# Autodesk Inventor assembly: PinBlock
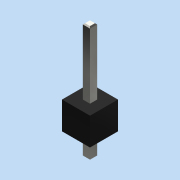
[picture p0: Inventor's stored thumbnail of the model, 180x180]
Saved by Autodesk Inventor 2017 (Build 210142000, 142)
## iProperties
Created: 2017-01-25
Part Number: PinBlock
Document SubType Name: Assembly
Designer: techn
Author: techn
## Documents named in this file (3)
- D:\OneDrive\Documents\Other Projects\Submarine\CAD\midships\ElectronicsSection\ServoController\PinBlock.iam
- D:\OneDrive\Documents\Other Projects\Submarine\CAD\midships\ElectronicsSection\ServoController\Pin.ipt
- D:\OneDrive\Documents\Other Projects\Submarine\CAD\midships\ElectronicsSection\ServoController\PinBlock.ipt
## Components (2 placed, 2 different names)
1. Pin:1 — Mate:1, Mate:2, Flush:1
2. PinBlock:1 — Mate:1, Mate:2, Flush:1
## Relationships (3: Mate 2, Flush 1)
- Mate:1: Pin:1 ↔ PinBlock:1
- Mate:2: Pin:1 ↔ PinBlock:1
- Flush:1 (-2 mm): Pin:1 ↔ PinBlock:1
